# Autodesk Inventor assembly: PD Rev3 Assembly
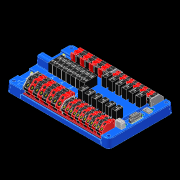
[picture p0: Inventor's stored thumbnail of the model, 180x180]
Saved by Autodesk Inventor 2012 (Build 160160000, 160)
## iProperties
Company: Team 801
Created: 2008-05-31
Part Number: PD Rev3 Assembly
Document SubType Name: Assembly
Designer: Jeffrey M
Catalog Web Link: www.team801.org
Author: Jeffrey M
## Documents named in this file (6)
- Z:\UserData\Documents\Inventor\team1885frc\Electronics\PowerDistributionBoard\elc_Power_Distro_inv.iam
- Z:\UserData\Documents\Inventor\team1885frc\Electronics\PowerDistributionBoard\PD Rev3 Bottom.ipt
- Z:\UserData\Documents\Inventor\team1885frc\Electronics\PowerDistributionBoard\PD Rev3 PCB.iam
- Z:\UserData\Documents\Inventor\team1885frc\Electronics\PowerDistributionBoard\PD Rev3 Top.ipt
- Z:\UserData\Documents\Inventor\team1885frc\Electronics\PowerDistributionBoard\Wago 734-102.ipt
- Z:\UserData\Documents\Inventor\team1885frc\Electronics\PowerDistributionBoard\CTF040V8.iam
## Components (5 placed, 5 different names)
1. PD Rev3 Bottom:1 — Mate:1, Mate:2, Mate:3, Mate:4, Mate:5
2. CTF040V8:1 [sub-assembly] — Mate:8, Mate:9, Mate:10
3. PD Rev3 PCB:1 [sub-assembly] — Mate:1, Mate:2, Mate:6, Mate:7, Mate:8, Mate:9, Mate:10, Flush:1
4. PD Rev3 Top:1 — Mate:3, Mate:4, Mate:5, Flush:1
5. 734-102:1 — Mate:6, Mate:7
## Relationships (11: Mate 10, Flush 1)
- Mate:1: PD Rev3 Bottom:1 ↔ PD Rev3 PCB:1
- Mate:2: PD Rev3 Bottom:1 ↔ PD Rev3 PCB:1
- Mate:3: PD Rev3 Bottom:1 ↔ PD Rev3 Top:1
- Mate:4: PD Rev3 Bottom:1 ↔ PD Rev3 Top:1
- Mate:5: PD Rev3 Bottom:1 ↔ PD Rev3 Top:1
- Mate:6: PD Rev3 PCB:1 ↔ 734-102:1
- Mate:7: PD Rev3 PCB:1 ↔ 734-102:1
- Mate:8: CTF040V8:1 ↔ PD Rev3 PCB:1
- Mate:9: CTF040V8:1 ↔ PD Rev3 PCB:1
- Mate:10: CTF040V8:1 ↔ PD Rev3 PCB:1
- Flush:1: PD Rev3 PCB:1 ↔ PD Rev3 Top:1
